# Autodesk Inventor assembly: AXp2p
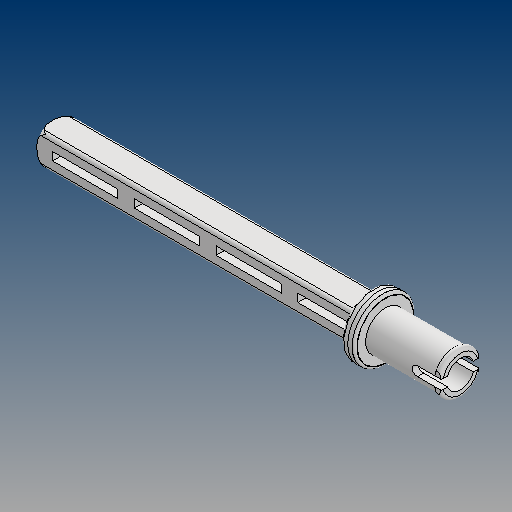
[picture p0: Inventor's stored thumbnail of the model, 512x512]
Saved by Autodesk Inventor 2020 (Build 240168000, 168)
## iProperties
Created: 2019-05-09
Part Number: AXp2p
Document SubType Name: Assembly
Designer: Varga Daniel
Author: Varga Daniel
## Documents named in this file (6)
- C:\!_Dani\!_cloud\OneDrive\!_munka\Revolution\StructuralParts\Axles\AXpXp\AXp4p.iam
- C:\!_Dani\!_cloud\OneDrive\!_munka\Revolution\StructuralParts\Connector pins\Connector_pin_base\Connector_pin_base_single_no_anti_skid.ipt
- C:\!_Dani\!_cloud\OneDrive\!_munka\Revolution\StructuralParts\Connector pins\Connector_pin_base.ipt
- C:\!_Dani\!_cloud\OneDrive\!_munka\Revolution\StructuralParts\Axles\Axle_collar.ipt
- C:\!_Dani\!_cloud\OneDrive\!_munka\Revolution\StructuralParts\Axles\One_sided_axle_base\One_sided_axle_base-40.ipt
- C:\!_Dani\!_cloud\OneDrive\!_munka\Revolution\StructuralParts\Axles\One_sided_axle_base.ipt
## Components (3 placed, 3 different names)
1. Connector_pin_base_single_no_anti_skid:1 — Mate:3, Mate:4, Flush:2, Flush:5, Flush:6
2. Axle_collar:1 — Mate:5, Mate:6, Flush:3
3. One_sided_axle_base-40:1 — Flush:4, Flush:5, Flush:6
## Relationships (9: Flush 5, Mate 4)
- Mate:3: Connector_pin_base_single_no_anti_skid:1
- Mate:4: Connector_pin_base_single_no_anti_skid:1
- Flush:2: Connector_pin_base_single_no_anti_skid:1
- Mate:5: Axle_collar:1
- Mate:6: Axle_collar:1
- Flush:3: Axle_collar:1
- Flush:4: One_sided_axle_base-40:1
- Flush:5: Connector_pin_base_single_no_anti_skid:1 ↔ One_sided_axle_base-40:1
- Flush:6: Connector_pin_base_single_no_anti_skid:1 ↔ One_sided_axle_base-40:1
